# Autodesk Inventor assembly: sensingtangible_large_touch
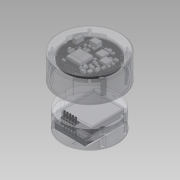
[picture p0: Inventor's stored thumbnail of the model, 180x180]
Saved by Autodesk Inventor 2015 SP2 (Build 190223200, 223)
## iProperties
Created: 2015-04-11
Part Number: sensingtangible_large_touch
Document SubType Name: Assembly
Designer: Mathieu
Author: Mathieu
## Documents named in this file (4)
- D:\Users\Mathieu\Desktop\SmartTokens\SmartTokens\Inventor Files\smart_token.iam
- D:\Users\Mathieu\Desktop\SmartTokens\SmartTokens\Inventor Files\top.ipt
- D:\Users\Mathieu\Desktop\SmartTokens\SmartTokens\Inventor Files\battery_block.iam
- D:\Users\Mathieu\Desktop\SmartTokens\SmartTokens\Inventor Files\pcb.ipt
## Components (3 placed, 3 different names)
1. top:1 — Mate:10, Mate:11, Mate:12
2. pcb:1 — Mate:12
3. battery_block:1 [sub-assembly] — Mate:10, Mate:11
## Relationships (3: Mate 3)
- Mate:10: top:1 ↔ battery_block:1
- Mate:11: top:1 ↔ battery_block:1
- Mate:12: top:1 ↔ pcb:1
